# Autodesk Inventor assembly: SlidingDoor
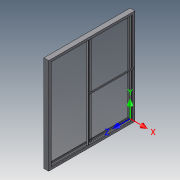
[picture p0: Inventor's stored thumbnail of the model, 180x180]
Saved by Autodesk Inventor 2018.3 (Build 223284000, 284)
## iProperties
Created: 2019-11-06
Part Number: SlidingDoor
Document SubType Name: Assembly
Designer: MattBussey
RuleStatus: InUse
Author: MattBussey
## Documents named in this file (3)
- C:\AVAInvAPI\Workspace\Assets\SlidingDoor.iam
- C:\AVAInvAPI\Workspace\Assets\SlidingDoorFrame.ipt
- C:\AVAInvAPI\Workspace\Assets\SlidingDoorPanel.ipt
## Components (2 placed, 2 different names)
1. SlidingDoorFrame:1 — Mate:1, FloorMate, MateLeft, MateInterior, MateRight, MateExterior
2. SlidingDoorPanel:1 — FloorMate, MateLeft, MateInterior, MateRight, MateExterior
## Relationships (6: Mate 6)
- Mate:1: SlidingDoorFrame:1
- FloorMate [Mate]: SlidingDoorFrame:1 ↔ SlidingDoorPanel:1
- MateLeft: SlidingDoorFrame:1 ↔ SlidingDoorPanel:1
- MateInterior: SlidingDoorFrame:1 ↔ SlidingDoorPanel:1
- MateRight: SlidingDoorFrame:1 ↔ SlidingDoorPanel:1
- MateExterior: SlidingDoorFrame:1 ↔ SlidingDoorPanel:1
## Named parameters: Width = 1828.8 mm, Depth = 101.6 mm, Height = 2032 mm
